# Autodesk Inventor assembly: POM_T5_20
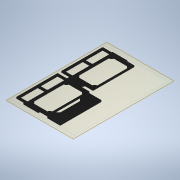
[picture p0: Inventor's stored thumbnail of the model, 180x180]
Saved by Autodesk Inventor 2020 (Build 240168000, 168)
## iProperties
Created: 2021-08-27
Part Number: POM_T5_20
Document SubType Name: Assembly
Designer: Masato
Author: Masato
## Documents named in this file (4)
- C:\Inventor\SUSTAINA-OP\Cam\POM_T5_20.iam
- C:\Inventor\SUSTAINA-OP\Cam\DisposableBoard.ipt
- C:\Inventor\SUSTAINA-OP\UpperBody\Cockpit\Cockpit_circuit_board_frame.ipt
- C:\Inventor\SUSTAINA-OP\UpperBody\Cockpit\Cockpit_battery_back_door.ipt
## Components (4 placed, 3 different names)
1. DisposableBoard:1 — メイト:2, メイト:1, フラッシュ:1, フラッシュ:2, メイト:20, メイト:21, フラッシュ:3, フラッシュ:4
2. Cockpit_battery_back_door:1 — メイト:21, フラッシュ:5, メイト:22
3. Cockpit_circuit_board_frame:1 — メイト:20, フラッシュ:3, フラッシュ:4, フラッシュ:5, メイト:22
4. Cockpit_circuit_board_frame:2
## Component patterns: (2 elements, first: Cockpit_circuit_board_frame:1)
## Relationships (10: Mate 5, Flush 5)
- メイト:2 [Mate]: DisposableBoard:1
- メイト:1 [Mate]: DisposableBoard:1
- フラッシュ:1 [Flush]: DisposableBoard:1
- フラッシュ:2 [Flush]: DisposableBoard:1
- メイト:20 [Mate]: DisposableBoard:1 ↔ Cockpit_circuit_board_frame:1
- メイト:21 [Mate]: DisposableBoard:1 ↔ Cockpit_battery_back_door:1
- フラッシュ:3 [Flush] (2 mm): DisposableBoard:1 ↔ Cockpit_circuit_board_frame:1
- フラッシュ:4 [Flush] (2 mm): DisposableBoard:1 ↔ Cockpit_circuit_board_frame:1
- フラッシュ:5 [Flush]: Cockpit_battery_back_door:1 ↔ Cockpit_circuit_board_frame:1
- メイト:22 [Mate] (2.5 mm): Cockpit_battery_back_door:1 ↔ Cockpit_circuit_board_frame:1
